# Autodesk Inventor assembly: BB-100
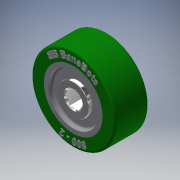
[picture p0: Inventor's stored thumbnail of the model, 180x180]
Saved by Autodesk Inventor 2019.4 (Build 234330000, 330)
## iProperties
Created: 2020-01-28
Part Number: BB-100
Document SubType Name: Assembly
Designer: mavericks
Author: mavericks
## Documents named in this file (3)
- T:\EIT\2020 Infinite Recharge\2020 ROBOT\COMMON PARTS\BANEBOTS\BB-100.iam
- T:\EIT\2020 Infinite Recharge\2020 ROBOT\COMMON PARTS\BANEBOTS\T81H_3_8_HEXT81H-HS61.ipt
- T:\EIT\2020 Infinite Recharge\2020 ROBOT\COMMON PARTS\BANEBOTS\T81P-20.ipt
## Components (2 placed, 2 different names)
1. T81H_3_8_HEXT81H-HS61:1 — Insert:1
2. T81P-20:1 — Insert:1
## Relationships (1: Insert 1)
- Insert:1: T81H_3_8_HEXT81H-HS61:1 ↔ T81P-20:1
